# Autodesk Inventor assembly: Assembly1
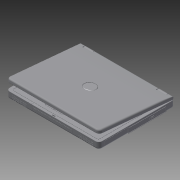
[picture p0: Inventor's stored thumbnail of the model, 180x180]
Saved by Autodesk Inventor 2015 (Build 190159000, 159)
## iProperties
Created: 2015-07-04
Part Number: Assembly1
Document SubType Name: Assembly
Designer: tsayman
Author: tsayman
## Documents named in this file (3)
- C:\Users\Owner\Documents\GrabCAD\Driver Station\Imported Components\Assembly1.iam
- C:\Users\Owner\Documents\GrabCAD\Driver Station\Imported Components\Part2.ipt
- C:\Users\Owner\Documents\GrabCAD\Driver Station\Imported Components\Part4.ipt
## Components (2 placed, 2 different names)
1. Part2:1 — Mate:1, Mate:2
2. Part4:1 — Mate:1, Mate:2
## Relationships (2: Mate 2)
- Mate:1: Part2:1 ↔ Part4:1
- Mate:2: Part2:1 ↔ Part4:1
